# Autodesk Inventor assembly: 10inchassemblycarbonarms
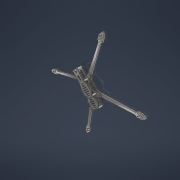
[picture p0: Inventor's stored thumbnail of the model, 180x180]
Saved by Autodesk Inventor 2021 (Build 250183000, 183)
## iProperties
Created: 2020-04-30
Part Number: 10inchassemblycarbonarms
Document SubType Name: Assembly
Designer: Logan
Mass: 95.3556 g
Surface Area: 673.203 cm^2
Volume: 95.3556 cm^3
Density: 1 g/cm^3
Author: Logan
## Documents named in this file (10)
- D:\Users\Logan\Downloads\10inchassemblycarbonarms.iam
- D:\Users\Logan\Downloads\10inchbottomplate.ipt
- D:\Users\Logan\Downloads\10inchbraceplate.ipt
- D:\Users\Logan\Downloads\standoff20mm.ipt
- D:\Users\Logan\Downloads\10inchtopplate.ipt
- D:\Users\Logan\Downloads\mc3525.ipt
- D:\Users\Logan\Downloads\10inchfrontarm.ipt
- D:\Users\Logan\Downloads\10inchreararm.ipt
- D:\Users\Logan\Downloads\cnhl1100.ipt
- D:\Users\Logan\Downloads\cnhl3000.ipt
## Components (22 placed, 9 different names)
1. 10inchbottomplate:1 — Mate:30, Mate:31, Mate:32, Mate:33, Mate:34, Mate:35, Mate:36, Mate:37, Mate:38, Mate:39, Mate:40, Mate:41, Mate:42, Mate:43, Mate:44, Mate:45, Mate:49, Mate:50, Mate:51, Mate:52, Mate:53, Mate:54, Mate:55, Mate:56, Mate:57, Mate:58, Mate:59, Mate:60
2. standoff20mm:1 — Mate:30, Mate:45, Mate:47
3. standoff20mm:2 — Mate:31, Mate:44
4. standoff20mm:3 — Mate:32, Mate:43
5. standoff20mm:4 — Mate:33, Mate:42, Mate:46
6. standoff20mm:5 — Mate:34, Mate:40
7. standoff20mm:6 — Mate:35, Mate:41
8. standoff20mm:7 — Mate:36, Mate:39
9. standoff20mm:8 — Mate:37, Mate:38, Mate:48
10. 10inchtopplate:1 — Mate:46, Mate:47, Mate:48, Mate:72, Mate:73, Flush:2, Mate:74, Flush:3
11. 10inchfrontarm:1 — Mate:49, Mate:50, Mate:51, Mate:61, Mate:62, Mate:67, Mate:69
12. 10inchfrontarm:2 — Mate:52, Mate:53, Mate:54, Mate:63, Mate:64, Mate:68
13. 10inchreararm:1 — Mate:58, Mate:59, Mate:60, Mate:66, Mate:70
14. 10inchreararm:2 — Mate:55, Mate:56, Mate:57, Mate:65, Mate:71
15. 10inchbraceplate:1 — Mate:61, Mate:62, Mate:63
16. mc3525:1 — Mate:67, Mate:69
17. mc3525:2 — Mate:66, Mate:70
18. mc3525:3 — Mate:65, Mate:71
19. mc3525:4 — Mate:64, Mate:68
20. cnhl1100:1 — Mate:73, Flush:2
21. cnhl1100:2 — Mate:72
22. cnhl3000:1 — Mate:74, Flush:3
## Relationships (47: Mate 45, Flush 2)
- Mate:30: 10inchbottomplate:1 ↔ standoff20mm:1
- Mate:31: 10inchbottomplate:1 ↔ standoff20mm:2
- Mate:32: 10inchbottomplate:1 ↔ standoff20mm:3
- Mate:33: 10inchbottomplate:1 ↔ standoff20mm:4
- Mate:34: 10inchbottomplate:1 ↔ standoff20mm:5
- Mate:35: 10inchbottomplate:1 ↔ standoff20mm:6
- Mate:36: 10inchbottomplate:1 ↔ standoff20mm:7
- Mate:37: 10inchbottomplate:1 ↔ standoff20mm:8
- Mate:38: 10inchbottomplate:1 ↔ standoff20mm:8
- Mate:39: 10inchbottomplate:1 ↔ standoff20mm:7
- Mate:40: 10inchbottomplate:1 ↔ standoff20mm:5
- Mate:41: 10inchbottomplate:1 ↔ standoff20mm:6
- Mate:42: 10inchbottomplate:1 ↔ standoff20mm:4
- Mate:43: 10inchbottomplate:1 ↔ standoff20mm:3
- Mate:44: 10inchbottomplate:1 ↔ standoff20mm:2
- Mate:45: 10inchbottomplate:1 ↔ standoff20mm:1
- Mate:46: standoff20mm:4 ↔ 10inchtopplate:1
- Mate:47: standoff20mm:1 ↔ 10inchtopplate:1
- Mate:48: standoff20mm:8 ↔ 10inchtopplate:1
- Mate:49: 10inchbottomplate:1 ↔ 10inchfrontarm:1
- Mate:50: 10inchbottomplate:1 ↔ 10inchfrontarm:1
- Mate:51: 10inchbottomplate:1 ↔ 10inchfrontarm:1
- Mate:52: 10inchbottomplate:1 ↔ 10inchfrontarm:2
- Mate:53: 10inchbottomplate:1 ↔ 10inchfrontarm:2
- Mate:54: 10inchbottomplate:1 ↔ 10inchfrontarm:2
- Mate:55: 10inchbottomplate:1 ↔ 10inchreararm:2
- Mate:56: 10inchbottomplate:1 ↔ 10inchreararm:2
- Mate:57: 10inchbottomplate:1 ↔ 10inchreararm:2
- Mate:58: 10inchbottomplate:1 ↔ 10inchreararm:1
- Mate:59: 10inchbottomplate:1 ↔ 10inchreararm:1
- Mate:60: 10inchbottomplate:1 ↔ 10inchreararm:1
- Mate:61: 10inchfrontarm:1 ↔ 10inchbraceplate:1
- Mate:62: 10inchfrontarm:1 ↔ 10inchbraceplate:1
- Mate:63: 10inchfrontarm:2 ↔ 10inchbraceplate:1
- Mate:64: 10inchfrontarm:2 ↔ mc3525:4
- Mate:65: 10inchreararm:2 ↔ mc3525:3
- Mate:66: 10inchreararm:1 ↔ mc3525:2
- Mate:67: 10inchfrontarm:1 ↔ mc3525:1
- Mate:68: 10inchfrontarm:2 ↔ mc3525:4
- Mate:69: 10inchfrontarm:1 ↔ mc3525:1
- Mate:70: 10inchreararm:1 ↔ mc3525:2
- Mate:71: 10inchreararm:2 ↔ mc3525:3
- Mate:72: 10inchtopplate:1 ↔ cnhl1100:2
- Mate:73: 10inchtopplate:1 ↔ cnhl1100:1
- Flush:2 (-10 mm): 10inchtopplate:1 ↔ cnhl1100:1
- Mate:74: 10inchtopplate:1 ↔ cnhl3000:1
- Flush:3 (3 mm): 10inchtopplate:1 ↔ cnhl3000:1
